# Autodesk Inventor assembly: full_ring_2
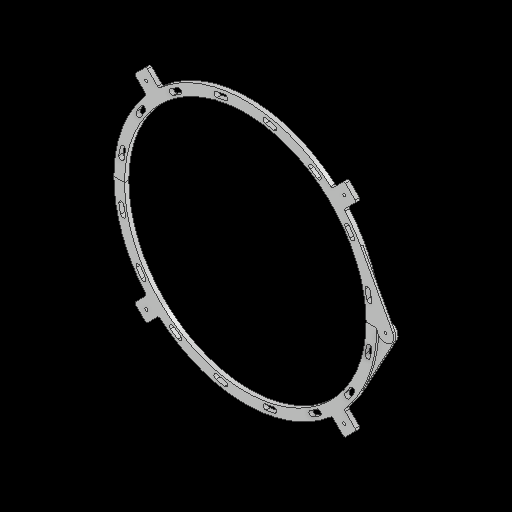
[picture p0: Inventor's stored thumbnail of the model, 512x512]
Saved by Autodesk Inventor 2026.1 (Build 301233000, 233)
## iProperties
Created: 2025-09-24
Part Number: full_ring_2
Document SubType Name: Assembly
Designer: drago
Author: drago
## Documents named in this file (2)
- C:\Users\drago\Desktop\_QIST4500_Multidisciplinary_Team_Project\Proteox MX magnet positioner CAD\full_ring_2.iam
- C:\Users\drago\Desktop\_QIST4500_Multidisciplinary_Team_Project\Proteox MX magnet positioner CAD\gantry_frame\half_ring_2.ipt
## Components (2 placed, 1 different names)
1. half_ring_2:1 — Mate:1, Mate:2, Mate:4, Mate:5, Mate:6
2. half_ring_2:2 — Mate:2, Mate:5, Mate:6
## Relationships (5: Mate 5)
- Mate:1: half_ring_2:1
- Mate:2: half_ring_2:1 ↔ half_ring_2:2
- Mate:4: half_ring_2:1
- Mate:5: half_ring_2:1 ↔ half_ring_2:2
- Mate:6: half_ring_2:1 ↔ half_ring_2:2
